# Autodesk Inventor assembly: pto front sprockets
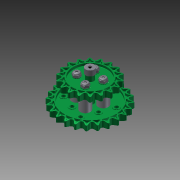
[picture p0: Inventor's stored thumbnail of the model, 180x180]
Saved by Autodesk Inventor 2014 SP1 (Build 180222100, 222)
## iProperties
Created: 2014-02-23
Part Number: pto front sprockets
Document SubType Name: Assembly
Designer: Ryan
Author: Ryan
## Documents named in this file (8)
- C:\Users\Ryan\Desktop\sw\toss up 4th robot\drive\pto front sprockets.iam
- C:\Users\Ryan\Desktop\sw\lib\Aperture VEX CAD Library\Sprockets\green\High Strength 24-Tooth Sprocket.ipt
- C:\Users\Ryan\Desktop\sw\lib\Aperture VEX CAD Library\Sprockets\green\High Strength 18-Tooth Sprocket.ipt
- C:\Users\Ryan\Desktop\sw\lib\Aperture VEX CAD Library\Hardware\Shaft Collar.ipt
- C:\Users\Ryan\Desktop\sw\lib\Aperture VEX CAD Library\Spacers\SPACER-0500-0125.ipt
- C:\Users\Ryan\Desktop\sw\lib\Aperture VEX CAD Library\Spacers\SPACER-0500-0375.ipt
- C:\Users\Ryan\Desktop\sw\lib\Aperture VEX CAD Library\Hardware\8-32\8-32_1.125.ipt
- C:\Users\Ryan\Desktop\sw\lib\Aperture VEX CAD Library\Hardware\8-32\8-32 nylock.ipt
## Components (25 placed, 7 different names)
1. High Strength 24-Tooth Sprocket:1 — Mate:1, Mate:2, Mate:3, Mate:6, Mate:9, Mate:10, Mate:15
2. High Strength 18-Tooth Sprocket:1 — Mate:3, Mate:4, Mate:5, Mate:6, Mate:7, Mate:8, Mate:11, Mate:13
3. Shaft Collar:1 — Mate:4, Mate:5
4. SPACER-0500-0125:1 — Mate:1, Mate:2
5. SPACER-0500-0375:1 — Mate:7, Mate:8
6. 8-32_1.125:1 — Mate:9, Mate:10, Mate:11, Mate:12, Mate:14, Mate:16
7. SPACER-0500-0375:3 — Mate:16, Mate:17, Mate:18, Mate:19
8. SPACER-0500-0375:2 — Mate:14, Mate:15, Mate:17
9. SPACER-0500-0125:2 — Mate:18, Mate:19
10. 8-32 nylock:1 — Mate:12, Mate:13
11. 8-32_1.125:2
12. SPACER-0500-0375:4
13. SPACER-0500-0375:5
14. SPACER-0500-0125:3
15. 8-32 nylock:2
16. 8-32_1.125:3
17. SPACER-0500-0375:6
18. SPACER-0500-0375:7
19. SPACER-0500-0125:4
20. 8-32 nylock:3
21. 8-32_1.125:4
22. SPACER-0500-0375:8
23. SPACER-0500-0375:9
24. SPACER-0500-0125:5
25. 8-32 nylock:4
## Component patterns: (4 elements, first: 8-32_1.125:1 + SPACER-0500-0375:3 + SPACER-0500-0375:2 + SPACER-0500-0125:2 + 8-32 nylock:1)
## Relationships (19: Mate 19)
- Mate:1: High Strength 24-Tooth Sprocket:1 ↔ SPACER-0500-0125:1
- Mate:2: High Strength 24-Tooth Sprocket:1 ↔ SPACER-0500-0125:1
- Mate:3 (9.271 mm): High Strength 24-Tooth Sprocket:1 ↔ High Strength 18-Tooth Sprocket:1
- Mate:4: High Strength 18-Tooth Sprocket:1 ↔ Shaft Collar:1
- Mate:5: High Strength 18-Tooth Sprocket:1 ↔ Shaft Collar:1
- Mate:6: High Strength 24-Tooth Sprocket:1 ↔ High Strength 18-Tooth Sprocket:1
- Mate:7: High Strength 18-Tooth Sprocket:1 ↔ SPACER-0500-0375:1
- Mate:8: High Strength 18-Tooth Sprocket:1 ↔ SPACER-0500-0375:1
- Mate:9: High Strength 24-Tooth Sprocket:1 ↔ 8-32_1.125:1
- Mate:10: High Strength 24-Tooth Sprocket:1 ↔ 8-32_1.125:1
- Mate:11: High Strength 18-Tooth Sprocket:1 ↔ 8-32_1.125:1
- Mate:12: 8-32_1.125:1 ↔ 8-32 nylock:1
- Mate:13: High Strength 18-Tooth Sprocket:1 ↔ 8-32 nylock:1
- Mate:14: 8-32_1.125:1 ↔ SPACER-0500-0375:2
- Mate:15: High Strength 24-Tooth Sprocket:1 ↔ SPACER-0500-0375:2
- Mate:16: 8-32_1.125:1 ↔ SPACER-0500-0375:3
- Mate:17: SPACER-0500-0375:3 ↔ SPACER-0500-0375:2
- Mate:18: SPACER-0500-0375:3 ↔ SPACER-0500-0125:2
- Mate:19: SPACER-0500-0375:3 ↔ SPACER-0500-0125:2
